# Autodesk Inventor assembly: 15102898-16-A-0000
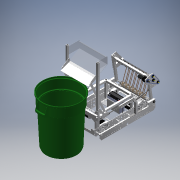
[picture p0: Inventor's stored thumbnail of the model, 180x180]
Saved by Autodesk Inventor 2017 (Build 210142000, 142)
## iProperties
Created: 2016-09-11
Part Number: 15102898-16-A-0000
Document SubType Name: Assembly
Designer: gus
Mass: 6306.62 g
Surface Area: 34906 cm^2
Volume: 6213.99 cm^3
Density: 1.01491 g/cm^3
Author: gus
## Documents named in this file (9)
- C:\Users\15102898\Documents\GitHub\bps-bunnybots2016-cad\Bunnybot-To_be_renamed\15102898-16-A-0000\15102898-16-A-0000.iam
- C:\Users\15102898\Documents\GitHub\bps-bunnybots2016-cad\Bunnybot-To_be_renamed\15102898-16-A-0000\15102898-16-A-0100\15102898-16-A-0100.iam
- C:\Users\15102898\Documents\GitHub\bps-bunnybots2016-cad\Bunnybot-To_be_renamed\15102898-16-A-0000\15102898-16-A-0200\15102898-16-A-0200.iam
- C:\Users\15102898\Documents\GitHub\bps-bunnybots2016-cad\Bunnybot-To_be_renamed\15102898-16-A-0000\15102898-16-A-0300\15102898-16-A-0300.iam
- C:\Users\15102898\Documents\GitHub\bps-bunnybots2016-cad\Bunnybot-To_be_renamed\15102898-16-A-0000\recycling bin\RECYCLING_CAN.ipt
- C:\Users\15102898\Documents\GitHub\bps-bunnybots2016-cad\Bunnybot-To_be_renamed\15102898-16-A-0000\15102898-16-A-0400\15102898-16-A-0400.iam
- C:\Users\15102898\Documents\GitHub\bps-bunnybots2016-cad\Bunnybot-To_be_renamed\15102898-16-A-0000\15102898-16-A-0300\15102898-16-P-0306.ipt
- C:\Users\15102898\Documents\GitHub\bps-bunnybots2016-cad\Bunnybot-To_be_renamed\15102898-16-A-0000\15102898-16-A-0300\15102898-16-P-0306_MIR.ipt
- C:\Users\15102898\Documents\GitHub\bps-bunnybots2016-cad\Bunnybot-To_be_renamed\15102898-16-A-0000\15102898-16-A-0500.iam
## Components (8 placed, 8 different names)
1. 15102898-16-A-0100:1 [sub-assembly] — Mate:1, Mate:3, Mate:4, Flush:1, Mate:5, Flush:2, Mate:6, Flush:3, Mate:7, Mate:8, Flush:5, Flush:10, Mate:10
2. 15102898-16-A-0200:1 [sub-assembly] — Mate:1, Mate:3, Mate:4
3. 15102898-16-A-0300:2 [sub-assembly] — Rotational:1
4. RECYCLING_CAN:1
5. 15102898-16-A-0400:1 [sub-assembly] — Mate:5, Flush:2, Mate:6
6. 15102898-16-P-0306:1 — Flush:3, Mate:7, Rotational:1, Mate:8, Flush:4, Flush:6
7. 15102898-16-P-0306_MIR:1 — Flush:4, Flush:5, Flush:6
8. 15102898-16-A-0500:1 [sub-assembly] — Flush:10, Mate:10
## Relationships (16: Mate 8, Flush 7, RevoluteJoint 1)
- Mate:1: 15102898-16-A-0100:1 ↔ 15102898-16-A-0200:1
- Mate:3 (34.925 mm): 15102898-16-A-0100:1 ↔ 15102898-16-A-0200:1
- Mate:4 (3.175 mm): 15102898-16-A-0100:1 ↔ 15102898-16-A-0200:1
- Flush:1 (-291.973 mm): 15102898-16-A-0100:1
- Mate:5: 15102898-16-A-0100:1 ↔ 15102898-16-A-0400:1
- Flush:2: 15102898-16-A-0100:1 ↔ 15102898-16-A-0400:1
- Mate:6: 15102898-16-A-0100:1 ↔ 15102898-16-A-0400:1
- Flush:3: 15102898-16-A-0100:1 ↔ 15102898-16-P-0306:1
- Mate:7: 15102898-16-A-0100:1 ↔ 15102898-16-P-0306:1
- Rotational:1 [RevoluteJoint]: 15102898-16-A-0300:2 ↔ 15102898-16-P-0306:1
- Mate:8: 15102898-16-A-0100:1 ↔ 15102898-16-P-0306:1
- Flush:4: 15102898-16-P-0306:1 ↔ 15102898-16-P-0306_MIR:1
- Flush:5: 15102898-16-A-0100:1 ↔ 15102898-16-P-0306_MIR:1
- Flush:6: 15102898-16-P-0306:1 ↔ 15102898-16-P-0306_MIR:1
- Flush:10: 15102898-16-A-0100:1 ↔ 15102898-16-A-0500:1
- Mate:10: 15102898-16-A-0100:1 ↔ 15102898-16-A-0500:1
